# Autodesk Inventor assembly: CenterWheel
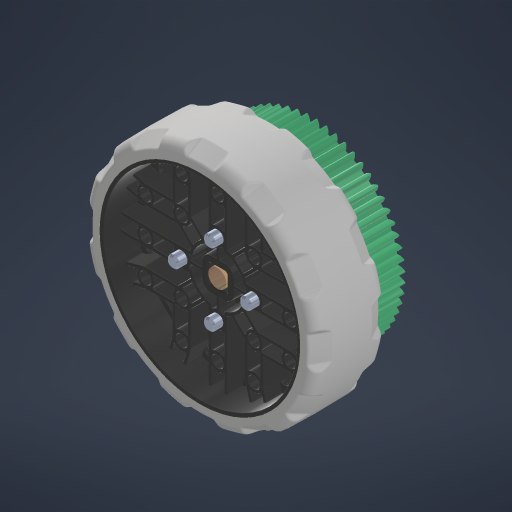
[picture p0: Inventor's stored thumbnail of the model, 512x512]
Saved by Autodesk Inventor 2023 (Build 270158000, 158)
## iProperties
Created: 2023-05-07
Part Number: CenterWheel
Document SubType Name: Assembly
Designer: alex
Author: alex
## Documents named in this file (8)
- C:\Users\alex\Documents\GitHub\4067X-Over-Under-CAD\Chassis\CenterWheel.iam
- C:\Users\alex\Documents\GitHub\4067X-Over-Under-CAD\VEX-CAD-Inventor\Structure\Standoff\Standoff .50.ipt
- C:\Users\alex\Documents\GitHub\4067X-Over-Under-CAD\VEX-CAD-Inventor\Structure\Standoff.ipt
- C:\Users\alex\Documents\GitHub\4067X-Over-Under-CAD\VEX-CAD-Inventor\Structure\Hardware\Screw Steel - Star.ipt
- C:\Users\alex\Documents\GitHub\4067X-Over-Under-CAD\VEX-CAD-Inventor\Structure\Hardware\Screw Steel - Star\SScrew Star Smooth 1.250.ipt
- C:\Users\alex\Documents\GitHub\4067X-Over-Under-CAD\VEX-CAD-Inventor\Motion\Gears\HS Gear\HS 60T Gear, No Insert Old.ipt
- C:\Users\alex\Documents\GitHub\4067X-Over-Under-CAD\VEX-CAD-Inventor\Motion\Wheels\Traction Wheel\3.25 Traction AS, No Insert.iam
- C:\Users\alex\Documents\GitHub\4067X-Over-Under-CAD\VEX-CAD-Inventor\Motion\Wheels\Traction Wheel.iam
## Components (10 placed, 4 different names)
1. HS 60T Gear, No Insert Old:1 — Insert:1, Insert:2, Insert:3, Insert:4, Insert:5, Insert:6, Insert:7, Insert:8
2. SScrew Star Smooth 1.250:1 — Insert:1
3. Standoff .50:1 — Insert:2, Insert:9
4. SScrew Star Smooth 1.250:2 — Insert:3
5. Standoff .50:2 — Insert:4, Insert:10
6. SScrew Star Smooth 1.250:3 — Insert:5
7. SScrew Star Smooth 1.250:4 — Insert:6
8. Standoff .50:3 — Insert:7
9. Standoff .50:4 — Insert:8
10. 3.25 Traction AS, No Insert:1 [sub-assembly] — Insert:9, Insert:10
## Relationships (10: Insert 10)
- Insert:1: HS 60T Gear, No Insert Old:1 ↔ SScrew Star Smooth 1.250:1
- Insert:2: HS 60T Gear, No Insert Old:1 ↔ Standoff .50:1
- Insert:3: HS 60T Gear, No Insert Old:1 ↔ SScrew Star Smooth 1.250:2
- Insert:4: HS 60T Gear, No Insert Old:1 ↔ Standoff .50:2
- Insert:5: HS 60T Gear, No Insert Old:1 ↔ SScrew Star Smooth 1.250:3
- Insert:6: HS 60T Gear, No Insert Old:1 ↔ SScrew Star Smooth 1.250:4
- Insert:7: HS 60T Gear, No Insert Old:1 ↔ Standoff .50:3
- Insert:8: HS 60T Gear, No Insert Old:1 ↔ Standoff .50:4
- Insert:9: Standoff .50:1 ↔ 3.25 Traction AS, No Insert:1
- Insert:10: Standoff .50:2 ↔ 3.25 Traction AS, No Insert:1
